# Autodesk Inventor assembly: AP1
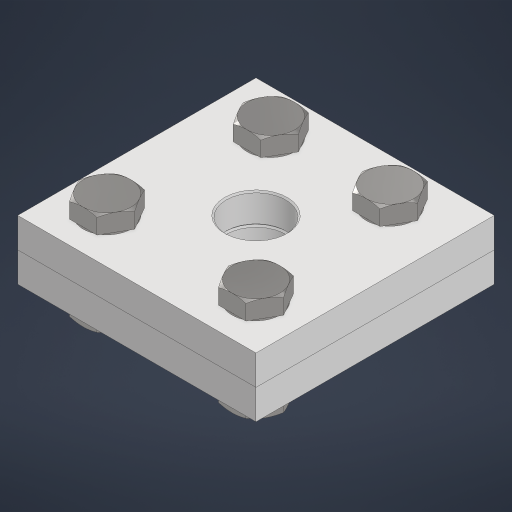
[picture p0: Inventor's stored thumbnail of the model, 512x512]
Saved by Autodesk Inventor 2024.3 (Build 283343000, 343)
## iProperties
Created: 2024-05-02
Part Number: AP1
Document SubType Name: Assembly
Designer: fablabadmin
Author: fablabadmin
## Documents named in this file (5)
- C:\Users\fablabadmin\Documents\_Benjamin_S\_3dCAD\HHVerkstad\AxlePlate\AP1.iam
- C:\Users\fablabadmin\Documents\_Benjamin_S\_3dCAD\HHVerkstad\AxlePlate\AP1-001.ipt
- C:\Users\fablabadmin\Documents\_Benjamin_S\_3dCAD\HHVerkstad\AxlePlate\AP1-002.ipt
- C:\Users\fablabadmin\Documents\Inventor\Content Center Files\R2024\en-US\AS 1110\AS 1110 - M10 x 30.ipt
- C:\Users\fablabadmin\Documents\Inventor\Content Center Files\R2024\en-US\AS 1112 (2)\AS 1112 - M10  Type 5.ipt
## Components (10 placed, 4 different names)
1. AP1-001:1 — Mate:1, Mate:2, Mate:3, Mate:4, Mate:5, Mate:7, Mate:9, Mate:11, Mate:13
2. AP1-002:1 — Mate:1, Mate:2, Mate:3, Mate:4, Mate:5, Insert:1, Insert:2, Insert:3, Insert:4
3. AS 1110 - Metric M10 x 30:1 — Insert:1, Mate:6
4. AS 1110 - Metric M10 x 30:2 — Insert:2, Mate:10
5. AS 1110 - Metric M10 x 30:3 — Insert:3, Mate:12
6. AS 1110 - Metric M10 x 30:4 — Insert:4, Mate:8
7. AS 1112 (2) - Metric M10  Type 5:1 — Mate:6, Mate:7
8. AS 1112 (2) - Metric M10  Type 5:2 — Mate:8, Mate:9
9. AS 1112 (2) - Metric M10  Type 5:3 — Mate:10, Mate:11
10. AS 1112 (2) - Metric M10  Type 5:4 — Mate:12, Mate:13
## Relationships (17: Mate 13, Insert 4)
- Mate:1: AP1-001:1 ↔ AP1-002:1
- Mate:2: AP1-001:1 ↔ AP1-002:1
- Mate:3: AP1-001:1 ↔ AP1-002:1
- Mate:4: AP1-001:1 ↔ AP1-002:1
- Mate:5: AP1-001:1 ↔ AP1-002:1
- Insert:1: AP1-002:1 ↔ AS 1110 - Metric M10 x 30:1
- Insert:2: AP1-002:1 ↔ AS 1110 - Metric M10 x 30:2
- Insert:3: AP1-002:1 ↔ AS 1110 - Metric M10 x 30:3
- Insert:4: AP1-002:1 ↔ AS 1110 - Metric M10 x 30:4
- Mate:6: AS 1110 - Metric M10 x 30:1 ↔ AS 1112 (2) - Metric M10  Type 5:1
- Mate:7: AP1-001:1 ↔ AS 1112 (2) - Metric M10  Type 5:1
- Mate:8: AS 1110 - Metric M10 x 30:4 ↔ AS 1112 (2) - Metric M10  Type 5:2
- Mate:9: AP1-001:1 ↔ AS 1112 (2) - Metric M10  Type 5:2
- Mate:10: AS 1110 - Metric M10 x 30:2 ↔ AS 1112 (2) - Metric M10  Type 5:3
- Mate:11: AP1-001:1 ↔ AS 1112 (2) - Metric M10  Type 5:3
- Mate:12: AS 1110 - Metric M10 x 30:3 ↔ AS 1112 (2) - Metric M10  Type 5:4
- Mate:13: AP1-001:1 ↔ AS 1112 (2) - Metric M10  Type 5:4
